# Autodesk Inventor assembly: GripperSidePlateFlipped
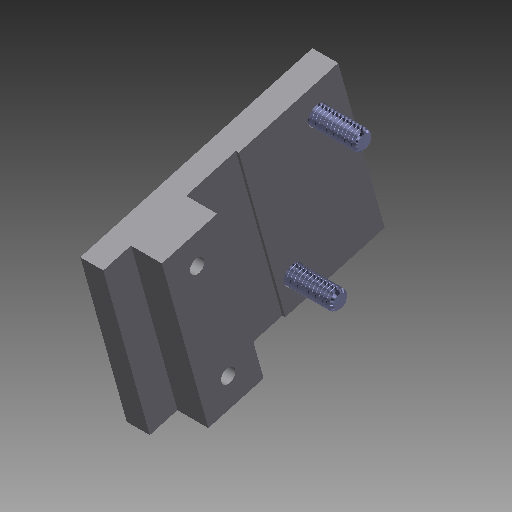
[picture p0: Inventor's stored thumbnail of the model, 512x512]
Saved by Autodesk Inventor 2019 (Build 230136000, 136)
## iProperties
Created: 2019-10-03
Part Number: GripperSidePlateFlipped
Document SubType Name: Assembly
Designer: james
Author: james
## Documents named in this file (5)
- F:\JimsDesign\Jims2020FTC\GripperSidePlateFlipped.iam
- F:\JimsDesign\Jims2020FTC\GripperSidePlateFlipped.ipt
- F:\JimsDesign\Library\McMaster\Screws\91771A196_18-8 SS FLAT HEAD PHILLIPS MACHINE SCREW.ipt
- F:\JimsDesign\Library\McMaster\Screws\91771A192_18-8 SS FLAT HEAD PHILLIPS MACHINE SCREW.ipt
- F:\JimsDesign\Jims2020FTC\GripperSliderBlock.ipt
## Components (6 placed, 4 different names)
1. GripperSidePlateFlipped:1 — Flush:1, Flush:2, Flush:3, Flush:4, Mate:5, Mate:7, Mate:8, Mate:9, Mate:10
2. 91771A196_18-8 SS FLAT HEAD PHILLIPS MACHINE SCREW:1 — Flush:3, Mate:8
3. 91771A196_18-8 SS FLAT HEAD PHILLIPS MACHINE SCREW:2 — Flush:2, Mate:7
4. 91771A192_18-8 SS FLAT HEAD PHILLIPS MACHINE SCREW:1 — Flush:1, Mate:10, Mate:12
5. 91771A192_18-8 SS FLAT HEAD PHILLIPS MACHINE SCREW:2 — Flush:4, Mate:9, Mate:11
6. GripperSliderBlock:1 — Mate:5, Mate:11, Mate:12
## Relationships (11: Mate 7, Flush 4)
- Flush:1: GripperSidePlateFlipped:1 ↔ 91771A192_18-8 SS FLAT HEAD PHILLIPS MACHINE SCREW:1
- Flush:2: GripperSidePlateFlipped:1 ↔ 91771A196_18-8 SS FLAT HEAD PHILLIPS MACHINE SCREW:2
- Flush:3: GripperSidePlateFlipped:1 ↔ 91771A196_18-8 SS FLAT HEAD PHILLIPS MACHINE SCREW:1
- Flush:4: GripperSidePlateFlipped:1 ↔ 91771A192_18-8 SS FLAT HEAD PHILLIPS MACHINE SCREW:2
- Mate:5: GripperSidePlateFlipped:1 ↔ GripperSliderBlock:1
- Mate:7: GripperSidePlateFlipped:1 ↔ 91771A196_18-8 SS FLAT HEAD PHILLIPS MACHINE SCREW:2
- Mate:8: GripperSidePlateFlipped:1 ↔ 91771A196_18-8 SS FLAT HEAD PHILLIPS MACHINE SCREW:1
- Mate:9: GripperSidePlateFlipped:1 ↔ 91771A192_18-8 SS FLAT HEAD PHILLIPS MACHINE SCREW:2
- Mate:10: GripperSidePlateFlipped:1 ↔ 91771A192_18-8 SS FLAT HEAD PHILLIPS MACHINE SCREW:1
- Mate:11: 91771A192_18-8 SS FLAT HEAD PHILLIPS MACHINE SCREW:2 ↔ GripperSliderBlock:1
- Mate:12: 91771A192_18-8 SS FLAT HEAD PHILLIPS MACHINE SCREW:1 ↔ GripperSliderBlock:1
